# Autodesk Inventor assembly: room
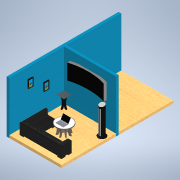
[picture p0: Inventor's stored thumbnail of the model, 180x180]
Saved by Autodesk Inventor 2022 (Build 260153000, 153)
## iProperties
Created: 2022-05-13
Part Number: room
Document SubType Name: Assembly
Designer: mihir
Author: mihir
## Documents named in this file (9)
- C:\Users\mihir\Documents\Personal\InventorBuilds\Room\room.iam
- C:\Users\mihir\Documents\Personal\InventorBuilds\Room\Wall.ipt
- C:\Users\mihir\Documents\Personal\InventorBuilds\Room\TV.ipt
- C:\Users\mihir\Documents\Personal\InventorBuilds\Room\couch.ipt
- C:\Users\mihir\Documents\Personal\InventorBuilds\Room\Table.ipt
- C:\Users\mihir\Documents\Personal\InventorBuilds\Room\Painting.ipt
- C:\Users\mihir\Documents\Personal\InventorBuilds\Laptop.iam
- C:\Users\mihir\Documents\Personal\InventorBuilds\Room\fan.ipt
- C:\Users\mihir\Documents\Personal\InventorBuilds\Room\stand.ipt
## Components (13 placed, 8 different names)
1. Wall:1 — Mate:2, Flush:2, Flush:3, Mate:3, Mate:12, Mate:13, Mate:17, Mate:20, Flush:11, Mate:21
2. Wall:2 — Mate:1, Flush:1, Flush:4, Mate:4, Mate:6, Mate:9, Mate:10, Flush:9, Mate:18, Flush:10
3. Wall:3 — Mate:1, Mate:2, Flush:1, Flush:2, Flush:3, Flush:4, Mate:5, Mate:7, Flush:5, Mate:8, Tangent:2, Mate:11, Mate:14, Flush:6, Flush:7, Mate:16, Flush:8, Mate:19, Flush:12, Flush:13
4. TV:1 — Mate:3, Mate:4, Mate:5
5. couch:1 — Mate:6, Mate:7, Flush:5, Tangent:1
6. Table:1 — Mate:8, Tangent:1, Tangent:2, Mate:15
7. Painting:1 — Mate:10, Mate:13, Mate:14
8. Painting:2 — Mate:9, Mate:11, Mate:12
9. Laptop:1 [sub-assembly] — Mate:15, Flush:6, Flush:7
10. fan:1 — Mate:16, Flush:8, Flush:9
11. stand:1 — Mate:17, Mate:18, Mate:19
12. Wall:4 — Flush:10, Mate:20, Flush:11
13. Wall:5 — Mate:21, Flush:12, Flush:13
## Relationships (36: Mate 21, Flush 13, Tangent 2)
- Mate:1: Wall:2 ↔ Wall:3
- Mate:2: Wall:1 ↔ Wall:3
- Flush:1: Wall:2 ↔ Wall:3
- Flush:2: Wall:1 ↔ Wall:3
- Flush:3: Wall:1 ↔ Wall:3
- Flush:4: Wall:2 ↔ Wall:3
- Mate:3: Wall:1 ↔ TV:1
- Mate:4 (15 mm): Wall:2 ↔ TV:1
- Mate:5 (50 mm): Wall:3 ↔ TV:1
- Mate:6 (10 mm): Wall:2 ↔ couch:1
- Mate:7: Wall:3 ↔ couch:1
- Flush:5 (10 mm): Wall:3 ↔ couch:1
- Mate:8: Wall:3 ↔ Table:1
- Tangent:1 (10 mm): couch:1 ↔ Table:1
- Tangent:2 (-65 mm): Wall:3 ↔ Table:1
- Mate:9: Wall:2 ↔ Painting:2
- Mate:10: Wall:2 ↔ Painting:1
- Mate:11 (60 mm): Wall:3 ↔ Painting:2
- Mate:12 (60 mm): Wall:1 ↔ Painting:2
- Mate:13 (30 mm): Wall:1 ↔ Painting:1
- Mate:14 (40 mm): Wall:3 ↔ Painting:1
- Mate:15: Table:1 ↔ Laptop:1
- Flush:6 (42.5 mm): Wall:3 ↔ Laptop:1
- Flush:7 (-50 mm): Wall:3 ↔ Laptop:1
- Mate:16: Wall:3 ↔ fan:1
- Flush:8 (85 mm): Wall:3 ↔ fan:1
- Flush:9 (95 mm): Wall:2 ↔ fan:1
- Mate:17: Wall:1 ↔ stand:1
- Mate:18: Wall:2 ↔ stand:1
- Mate:19: Wall:3 ↔ stand:1
- Flush:10: Wall:2 ↔ Wall:4
- Mate:20: Wall:1 ↔ Wall:4
- Flush:11: Wall:1 ↔ Wall:4
- Mate:21: Wall:1 ↔ Wall:5
- Flush:12: Wall:3 ↔ Wall:5
- Flush:13: Wall:3 ↔ Wall:5
